# Autodesk Inventor assembly: llanta trasera
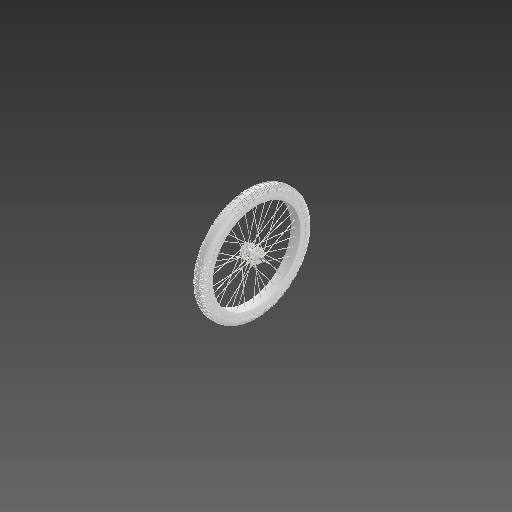
[picture p0: Inventor's stored thumbnail of the model, 512x512]
Saved by Autodesk Inventor 2021 (Build 250183000, 183)
## iProperties
Created: 2021-04-24
Part Number: llanta trasera
Document SubType Name: Assembly
Designer: j2seb
Author: j2seb
## Documents named in this file (6)
- C:\Users\maaro\Documents\UNAL\Automatización de Procesos de Manufactura\Github\Proyecto_APM\02 Inventor\llanta trasera.iam
- C:\Users\maaro\Documents\UNAL\Automatización de Procesos de Manufactura\Github\Proyecto_APM\02 Inventor\Ensamble_Llanta.iam
- C:\Users\maaro\Documents\UNAL\Automatización de Procesos de Manufactura\Github\Proyecto_APM\02 Inventor\eje manzana.ipt
- C:\Users\maaro\Documents\UNAL\Automatización de Procesos de Manufactura\Github\Proyecto_APM\02 Inventor\Transmision\Design Accelerator\Roller Chain Sprocket11.ipt
- C:\Users\maaro\Documents\UNAL\Automatización de Procesos de Manufactura\Github\Proyecto_APM\02 Inventor\retenedor_plato.ipt
- C:\Users\j2seb\OneDrive\Documents\Inventor\Content Center Files\R2021\es-ES\DIN 6923\DIN 6923 - M10 x 1,5.ipt
## Components (8 placed, 5 different names)
1. Ensamble_Llanta:1 [sub-assembly] — Coincidencia:1, Coincidencia:2, Nivelación:1, Coincidencia:3, Coincidencia:5, Nivelación:2, Coincidencia:7, Coincidencia:10, Coincidencia:12
2. eje manzana:1 — Coincidencia:1, Coincidencia:6, Coincidencia:9, Coincidencia:11
3. Roller Chain Sprocket1:1 — Coincidencia:2, Nivelación:1, Coincidencia:4
4. retenedor_plato:1 — Coincidencia:3, Coincidencia:4
5. retenedor_plato:2 — Coincidencia:6, Nivelación:2, Coincidencia:8
6. Roller Chain Sprocket1:2 — Coincidencia:5, Coincidencia:7, Coincidencia:8
7. DIN 6923 M10:1 — Coincidencia:9, Coincidencia:10
8. DIN 6923 M10:2 — Coincidencia:11, Coincidencia:12
## Relationships (14: Mate 12, Flush 2)
- Coincidencia:1 [Mate]: Ensamble_Llanta:1 ↔ eje manzana:1
- Coincidencia:2 [Mate]: Ensamble_Llanta:1 ↔ Roller Chain Sprocket1:1
- Nivelación:1 [Flush]: Ensamble_Llanta:1 ↔ Roller Chain Sprocket1:1
- Coincidencia:3 [Mate]: Ensamble_Llanta:1 ↔ retenedor_plato:1
- Coincidencia:4 [Mate]: Roller Chain Sprocket1:1 ↔ retenedor_plato:1
- Coincidencia:5 [Mate]: Ensamble_Llanta:1 ↔ Roller Chain Sprocket1:2
- Coincidencia:6 [Mate]: eje manzana:1 ↔ retenedor_plato:2
- Nivelación:2 [Flush]: Ensamble_Llanta:1 ↔ retenedor_plato:2
- Coincidencia:7 [Mate]: Ensamble_Llanta:1 ↔ Roller Chain Sprocket1:2
- Coincidencia:8 [Mate]: retenedor_plato:2 ↔ Roller Chain Sprocket1:2
- Coincidencia:9 [Mate]: eje manzana:1 ↔ DIN 6923 M10:1
- Coincidencia:10 [Mate] (5 mm): Ensamble_Llanta:1 ↔ DIN 6923 M10:1
- Coincidencia:11 [Mate]: eje manzana:1 ↔ DIN 6923 M10:2
- Coincidencia:12 [Mate] (5 mm): Ensamble_Llanta:1 ↔ DIN 6923 M10:2
